# Autodesk Inventor assembly: V4 - ASSEMBLY
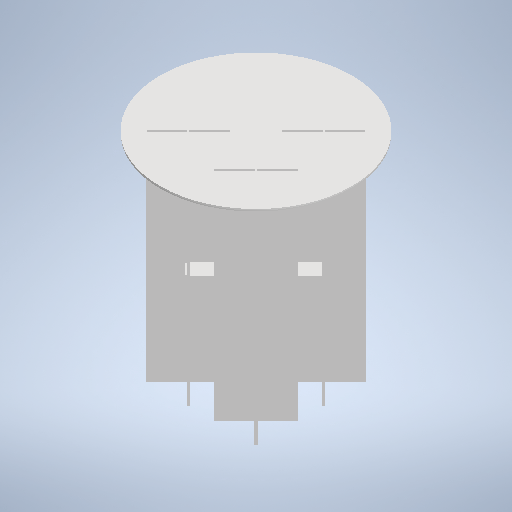
[picture p0: Inventor's stored thumbnail of the model, 512x512]
Saved by Autodesk Inventor 2025.2 (Build 292293000, 293)
## iProperties
Created: 2025-03-02
Part Number: V4 - ASSEMBLY
Document SubType Name: Assembly
Designer: Dylan
Mass: 427.641 g
Surface Area: 12805.5 cm^2
Volume: 2829.58 cm^3
Density: 0.151132 g/cm^3
Author: VRK99-0110
Title: Sustainable Chair_V4 - ASSEMBLY
Subject: Sustainable Chair Project
Comments: Version 4's final assembly.
## Documents named in this file (16)
- D:\GitHub\MMAE 232\Sustainable Chair\V4 - Assembly\---\Final Assembly\V4 - ASSEMBLY.iam
- D:\GitHub\MMAE 232\Sustainable Chair\V4 - Assembly\---\Final Assembly\Sustainable Chair_V2 - Seat.ipt
- D:\GitHub\MMAE 232\Sustainable Chair\V4 - Assembly\---\Final Assembly\Sustainable Chair_V2 - Leg(A)_1.ipt
- D:\GitHub\MMAE 232\Sustainable Chair\V4 - Assembly\---\Final Assembly\Sustainable Chair_V1 - Leg(B).ipt
- D:\GitHub\MMAE 232\Sustainable Chair\V4 - Assembly\---\Final Assembly\Sustainable Chair_V2 - Leg(A)_1_CPY.ipt
- D:\GitHub\MMAE 232\Sustainable Chair\V4 - Assembly\---\Final Assembly\Sustainable Chair_V1 - Leg(B)_CPY.ipt
- D:\GitHub\MMAE 232\Sustainable Chair\V4 - Assembly\---\Final Assembly\Sustainable Chair_V2 - Leg(A)_2.ipt
- D:\GitHub\MMAE 232\Sustainable Chair\V4 - Assembly\---\Final Assembly\Sustainable Chair_V2 - Leg(A)_2_CPY.ipt
- D:\GitHub\MMAE 232\Sustainable Chair\V4 - Assembly\---\Final Assembly\Sustainable Chair_V1 - Leg(B)_CPY1.ipt
- D:\GitHub\MMAE 232\Sustainable Chair\V4 - Assembly\---\Final Assembly\Sustainable Chair_V4 - Lateral Support.ipt
- C:\Users\Dylan\Documents\CAD\MMAE 232\Sustainable Chair\V4 - Assembly\V4 - ASSEMBLY\AIP\FEA\ezqprozfk.fins
- C:\Users\Dylan\Documents\CAD\MMAE 232\Sustainable Chair\V4 - Assembly\V4 - ASSEMBLY\AIP\FEA\ezqprozfk.fsat
- C:\Users\Dylan\Documents\CAD\MMAE 232\Sustainable Chair\V4 - Assembly\V4 - ASSEMBLY\AIP\FEA\ezqprozfk.ftes
- C:\Users\Dylan\Documents\CAD\MMAE 232\Sustainable Chair\V4 - Assembly\V4 - ASSEMBLY\AIP\FEA\ezqprozfk.fwiz
- C:\Users\Dylan\Documents\CAD\MMAE 232\Sustainable Chair\V4 - Assembly\V4 - ASSEMBLY\AIP\FEA\ezqprozk0.fmsh
- C:\Users\Dylan\Documents\CAD\MMAE 232\Sustainable Chair\V4 - Assembly\V4 - ASSEMBLY\AIP\FEA\ezqprozk1.fres
## Components (11 placed, 9 different names)
1. Sustainable Chair_V2 - Seat:1 — Mate:3, Mate:4, Flush:2, Mate:7, Mate:8, Flush:4, Mate:11, Mate:12, Flush:6, Mate:15, Mate:16, Flush:8
2. Sustainable Chair_V2 - Leg(A)_1:1 — Mate:1, Mate:2, Flush:1, Mate:4, Flush:2
3. Sustainable Chair_V1 - Leg(B):1 — Mate:1, Mate:2, Flush:1, Mate:3
4. Sustainable Chair_V2 - Leg(A)_1_CPY:1 — Flush:3, Mate:5, Mate:6, Mate:7, Flush:4, Mate:19, Mate:20, Flush:10
5. Sustainable Chair_V1 - Leg(B)_CPY:1 — Flush:3, Mate:5, Mate:6, Mate:8
6. Sustainable Chair_V2 - Leg(A)_2:1 — Mate:9, Mate:10, Flush:5, Mate:12, Mate:17, Mate:18, Flush:9
7. Sustainable Chair_V1 - Leg(B):2 — Mate:9, Mate:10, Flush:5, Mate:11, Flush:6
8. Sustainable Chair_V2 - Leg(A)_2_CPY:1 — Flush:7, Mate:13, Mate:14, Mate:16, Flush:8
9. Sustainable Chair_V1 - Leg(B)_CPY1:1 — Flush:7, Mate:13, Mate:14, Mate:15
10. Sustainable Chair_V4 - Lateral Support:1 — Mate:17, Mate:18, Flush:9
11. Sustainable Chair_V4 - Lateral Support:2 — Mate:19, Mate:20, Flush:10
## Relationships (30: Mate 20, Flush 10)
- Mate:1: Sustainable Chair_V2 - Leg(A)_1:1 ↔ Sustainable Chair_V1 - Leg(B):1
- Mate:2: Sustainable Chair_V2 - Leg(A)_1:1 ↔ Sustainable Chair_V1 - Leg(B):1
- Flush:1: Sustainable Chair_V2 - Leg(A)_1:1 ↔ Sustainable Chair_V1 - Leg(B):1
- Mate:3: Sustainable Chair_V2 - Seat:1 ↔ Sustainable Chair_V1 - Leg(B):1
- Mate:4: Sustainable Chair_V2 - Seat:1 ↔ Sustainable Chair_V2 - Leg(A)_1:1
- Flush:2: Sustainable Chair_V2 - Seat:1 ↔ Sustainable Chair_V2 - Leg(A)_1:1
- Flush:3: Sustainable Chair_V2 - Leg(A)_1_CPY:1 ↔ Sustainable Chair_V1 - Leg(B)_CPY:1
- Mate:5: Sustainable Chair_V2 - Leg(A)_1_CPY:1 ↔ Sustainable Chair_V1 - Leg(B)_CPY:1
- Mate:6: Sustainable Chair_V2 - Leg(A)_1_CPY:1 ↔ Sustainable Chair_V1 - Leg(B)_CPY:1
- Mate:7: Sustainable Chair_V2 - Seat:1 ↔ Sustainable Chair_V2 - Leg(A)_1_CPY:1
- Mate:8: Sustainable Chair_V2 - Seat:1 ↔ Sustainable Chair_V1 - Leg(B)_CPY:1
- Flush:4: Sustainable Chair_V2 - Seat:1 ↔ Sustainable Chair_V2 - Leg(A)_1_CPY:1
- Mate:9: Sustainable Chair_V2 - Leg(A)_2:1 ↔ Sustainable Chair_V1 - Leg(B):2
- Mate:10: Sustainable Chair_V2 - Leg(A)_2:1 ↔ Sustainable Chair_V1 - Leg(B):2
- Flush:5: Sustainable Chair_V2 - Leg(A)_2:1 ↔ Sustainable Chair_V1 - Leg(B):2
- Mate:11: Sustainable Chair_V2 - Seat:1 ↔ Sustainable Chair_V1 - Leg(B):2
- Mate:12: Sustainable Chair_V2 - Seat:1 ↔ Sustainable Chair_V2 - Leg(A)_2:1
- Flush:6: Sustainable Chair_V2 - Seat:1 ↔ Sustainable Chair_V1 - Leg(B):2
- Flush:7: Sustainable Chair_V2 - Leg(A)_2_CPY:1 ↔ Sustainable Chair_V1 - Leg(B)_CPY1:1
- Mate:13: Sustainable Chair_V2 - Leg(A)_2_CPY:1 ↔ Sustainable Chair_V1 - Leg(B)_CPY1:1
- Mate:14: Sustainable Chair_V2 - Leg(A)_2_CPY:1 ↔ Sustainable Chair_V1 - Leg(B)_CPY1:1
- Mate:15: Sustainable Chair_V2 - Seat:1 ↔ Sustainable Chair_V1 - Leg(B)_CPY1:1
- Mate:16: Sustainable Chair_V2 - Seat:1 ↔ Sustainable Chair_V2 - Leg(A)_2_CPY:1
- Flush:8: Sustainable Chair_V2 - Seat:1 ↔ Sustainable Chair_V2 - Leg(A)_2_CPY:1
- Mate:17: Sustainable Chair_V2 - Leg(A)_2:1 ↔ Sustainable Chair_V4 - Lateral Support:1
- Mate:18: Sustainable Chair_V2 - Leg(A)_2:1 ↔ Sustainable Chair_V4 - Lateral Support:1
- Flush:9: Sustainable Chair_V2 - Leg(A)_2:1 ↔ Sustainable Chair_V4 - Lateral Support:1
- Mate:19: Sustainable Chair_V2 - Leg(A)_1_CPY:1 ↔ Sustainable Chair_V4 - Lateral Support:2
- Mate:20: Sustainable Chair_V2 - Leg(A)_1_CPY:1 ↔ Sustainable Chair_V4 - Lateral Support:2
- Flush:10: Sustainable Chair_V2 - Leg(A)_1_CPY:1 ↔ Sustainable Chair_V4 - Lateral Support:2
## Named parameters: sa_0 = 60000
note: some values were not read from the file. Shown as the stored number, unit unknown: "sa_0".
